# Autodesk Inventor assembly: wood structure
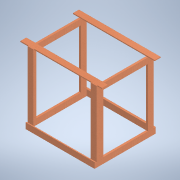
[picture p0: Inventor's stored thumbnail of the model, 180x180]
Saved by Autodesk Inventor 2020 (Build 240168000, 168)
## iProperties
Created: 2020-05-09
Part Number: wood structure
Document SubType Name: Assembly
Designer: kolbe
Author: kolbe
## Documents named in this file (7)
- C:\Users\kolbe\Documents\GitHub\Terrarium\wood structure.iam
- C:\Users\kolbe\Documents\GitHub\Terrarium\vertical beams.ipt
- C:\Users\kolbe\Documents\GitHub\Terrarium\length beams.ipt
- C:\Users\kolbe\Documents\GitHub\Terrarium\top beams.ipt
- C:\Users\kolbe\Documents\GitHub\Terrarium\back beam.ipt
- C:\Users\kolbe\Documents\GitHub\Terrarium\front beams.ipt
- C:\Users\kolbe\Documents\GitHub\Terrarium\door holder.ipt
## Components (14 placed, 6 different names)
1. vertical beams:1 — Mate:1, Mate:2, Mate:3, Mate:4, Mate:24
2. vertical beams:2 — Mate:5, Mate:6, Mate:13, Mate:14, Mate:19, Mate:22
3. length beams:1 — Mate:1, Mate:2, Mate:5
4. length beams:2 — Mate:3, Mate:4, Mate:6
5. vertical beams:3 — Mate:20, Mate:21, Mate:26
6. vertical beams:4 — Mate:15, Mate:16
7. length beams:3
8. length beams:4
9. top beams:1 — Mate:20, Mate:21, Mate:23, Mate:25
10. top beams:2 — Mate:19, Mate:22
11. back beam:1 — Mate:13, Mate:14, Mate:15, Mate:16
12. front beams:1 — Mate:23, Mate:24, Mate:27, Mate:28
13. front beams:2 — Mate:25, Mate:26
14. door holder:1 — Mate:27, Mate:28
## Relationships (26: Mate 26)
- Mate:1: vertical beams:1 ↔ length beams:1
- Mate:2: vertical beams:1 ↔ length beams:1
- Mate:3: vertical beams:1 ↔ length beams:2
- Mate:4: vertical beams:1 ↔ length beams:2
- Mate:5: vertical beams:2 ↔ length beams:1
- Mate:6: vertical beams:2 ↔ length beams:2
- [Mate]: vertical beams:3 ↔ length beams:3
- [Mate]: vertical beams:3 ↔ length beams:3
- [Mate]: vertical beams:3 ↔ length beams:4
- [Mate]: vertical beams:3 ↔ length beams:4
- [Mate]: vertical beams:4 ↔ length beams:3
- [Mate]: vertical beams:4 ↔ length beams:4
- Mate:13: vertical beams:2 ↔ back beam:1
- Mate:14: vertical beams:2 ↔ back beam:1
- Mate:15: vertical beams:4 ↔ back beam:1
- Mate:16: vertical beams:4 ↔ back beam:1
- Mate:19: vertical beams:2 ↔ top beams:2
- Mate:20: vertical beams:3 ↔ top beams:1
- Mate:21: vertical beams:3 ↔ top beams:1
- Mate:22: vertical beams:2 ↔ top beams:2
- Mate:23: top beams:1 ↔ front beams:1
- Mate:24: vertical beams:1 ↔ front beams:1
- Mate:25: top beams:1 ↔ front beams:2
- Mate:26: vertical beams:3 ↔ front beams:2
- Mate:27: front beams:1 ↔ door holder:1
- Mate:28: front beams:1 ↔ door holder:1
## Named parameters: d6_d2 = 0 mm, d7_d3 = 0 mm, d8_d4 = 0 mm, d9_d5 = 0 mm, d10_d0 = 0 mm, d11_d1 = 0 mm
